# Autodesk Inventor assembly: Robot
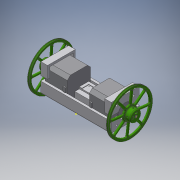
[picture p0: Inventor's stored thumbnail of the model, 180x180]
Saved by Autodesk Inventor 2019 (Build 230136000, 136)
## iProperties
Created: 2018-12-23
Part Number: Robot
Document SubType Name: Assembly
Designer: Martin
Author: Martin
## Documents named in this file (5)
- C:\Users\Martin\Projekte\Robby2\mechparts\Robot.iam
- C:\Users\Martin\Projekte\Robby2\mechparts\Motor BYGHW609.ipt
- C:\Users\Martin\Projekte\Robby2\mechparts\Wheel.ipt
- C:\Users\Martin\Projekte\Robby2\mechparts\Baseplate.ipt
- C:\Users\Martin\Projekte\Robby2\mechparts\Sideplate.ipt
## Components (7 placed, 4 different names)
1. Baseplate:1 — Mate:3, Mate:4, Mate:5, Mate:6, Mate:7, Mate:8
2. Sideplate:1 — Mate:9, Mate:10, Mate:11
3. Sideplate:2 — Mate:12, Mate:13, Mate:14
4. Motor BYGHW609:1 — Mate:1, Flush:1, Mate:3, Mate:4, Mate:5, Mate:9, Mate:10, Mate:11
5. Wheel:1 — Mate:1, Flush:1
6. Motor BYGHW609:2 — Mate:2, Flush:2, Mate:6, Mate:7, Mate:8, Mate:12, Mate:13, Mate:14
7. Wheel:2 — Mate:2, Flush:2
## Relationships (16: Mate 14, Flush 2)
- Mate:1: Motor BYGHW609:1 ↔ Wheel:1
- Flush:1 (0.5 mm): Motor BYGHW609:1 ↔ Wheel:1
- Mate:2: Motor BYGHW609:2 ↔ Wheel:2
- Flush:2 (0.5 mm): Motor BYGHW609:2 ↔ Wheel:2
- Mate:3: Baseplate:1 ↔ Motor BYGHW609:1
- Mate:4: Baseplate:1 ↔ Motor BYGHW609:1
- Mate:5: Baseplate:1 ↔ Motor BYGHW609:1
- Mate:6: Baseplate:1 ↔ Motor BYGHW609:2
- Mate:7: Baseplate:1 ↔ Motor BYGHW609:2
- Mate:8: Baseplate:1 ↔ Motor BYGHW609:2
- Mate:9: Sideplate:1 ↔ Motor BYGHW609:1
- Mate:10: Sideplate:1 ↔ Motor BYGHW609:1
- Mate:11: Sideplate:1 ↔ Motor BYGHW609:1
- Mate:12: Sideplate:2 ↔ Motor BYGHW609:2
- Mate:13: Sideplate:2 ↔ Motor BYGHW609:2
- Mate:14: Sideplate:2 ↔ Motor BYGHW609:2
